# Autodesk Inventor assembly: climber
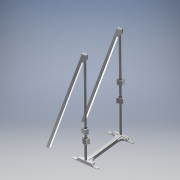
[picture p0: Inventor's stored thumbnail of the model, 180x180]
Saved by Autodesk Inventor 2019.4 (Build 234330000, 330)
## iProperties
Created: 2020-01-07
Part Number: climber
Document SubType Name: Assembly
Designer: Mark
Mass: 6066.58 g
Surface Area: 3692.19 cm^2
Volume: 1250.64 cm^3
Density: 4.85079 g/cm^3
Author: Mark
## Documents named in this file (8)
- C:\Users\Mark\Desktop\7738 Helion Engineering\7738-2020\Elevator Mechanism\climber.iam
- C:\Users\Mark\Desktop\7738 Helion Engineering\7738-2020\Elevator Mechanism\Extrusion Mid.ipt
- C:\Users\Mark\Desktop\7738 Helion Engineering\7738-2020\Elevator Mechanism\climber\Design Accelerator\Shaft2.iam
- C:\Users\Mark\Desktop\7738 Helion Engineering\7738-2020\Elevator Mechanism\scs20uu.ipt
- C:\Users\Mark\Desktop\jiagong\Base.ipt
- C:\Users\Mark\Desktop\7738 Helion Engineering\7738-2020\Elevator Mechanism\Standard Bracing.ipt
- C:\Users\Mark\Desktop\7738 Helion Engineering\7738-2020\Elevator Mechanism\Top Connector.ipt
- C:\Users\Mark\Desktop\7738 Helion Engineering\7738-2020\Elevator Mechanism\Elevator Support.ipt
## Components (17 placed, 7 different names)
1. Extrusion Mid:1 — Mate:10, Flush:3, Flush:4, Mate:12, Mate:13, Mate:16, Mate:19
2. Shaft:1 [sub-assembly] — Mate:3, Mate:4, Mate:7, Mate:8, Mate:20, Mate:21
3. Shaft:2 [sub-assembly] — Mate:1, Mate:2, Mate:6, Flush:1, Mate:26, Mate:27
4. scs20uu:1 — Mate:3
5. scs20uu:2 — Mate:1
6. scs20uu:3 — Mate:2
7. scs20uu:4 — Mate:4
8. Base:1 — Mate:6, Flush:1, Mate:9, Flush:2, Mate:10, Flush:3, Flush:4, Flush:5, Mate:11, Mate:17, Mate:18, Flush:10
9. Base:2 — Mate:7, Mate:8, Mate:9, Flush:2, Flush:5, Mate:14, Mate:15, Flush:6, Flush:7
10. Standard Bracing:1 — Mate:15, Mate:16
11. Standard Bracing:2 — Mate:13, Mate:14
12. Standard Bracing:3 — Mate:11, Mate:12
13. Standard Bracing:4 — Mate:17, Mate:18, Mate:19
14. Top Connector:1 — Mate:20, Flush:6, Mate:21, Flush:7, Mate:22, Flush:8, Mate:23
15. Elevator Support:1 — Mate:22, Flush:8, Mate:23
16. Top Connector:2 — Mate:26, Mate:27
17. Elevator Support:2 — Flush:10
## Relationships (36: Mate 26, Flush 10)
- Mate:1: Shaft:2 ↔ scs20uu:2
- Mate:2: Shaft:2 ↔ scs20uu:3
- Mate:3: Shaft:1 ↔ scs20uu:1
- Mate:4: Shaft:1 ↔ scs20uu:4
- Mate:6: Shaft:2 ↔ Base:1
- Flush:1: Shaft:2 ↔ Base:1
- Mate:7: Shaft:1 ↔ Base:2
- Mate:8: Shaft:1 ↔ Base:2
- Mate:9 (400 mm): Base:1 ↔ Base:2
- Flush:2: Base:1 ↔ Base:2
- Mate:10: Extrusion Mid:1 ↔ Base:1
- Flush:3: Extrusion Mid:1 ↔ Base:1
- Flush:4 (100 mm): Extrusion Mid:1 ↔ Base:1
- Flush:5: Base:1 ↔ Base:2
- Mate:11: Base:1 ↔ Standard Bracing:3
- Mate:12: Extrusion Mid:1 ↔ Standard Bracing:3
- Mate:13: Extrusion Mid:1 ↔ Standard Bracing:2
- Mate:14: Base:2 ↔ Standard Bracing:2
- Mate:15: Base:2 ↔ Standard Bracing:1
- Mate:16: Extrusion Mid:1 ↔ Standard Bracing:1
- Mate:17: Base:1 ↔ Standard Bracing:4
- Mate:18: Base:1 ↔ Standard Bracing:4
- Mate:19: Extrusion Mid:1 ↔ Standard Bracing:4
- Mate:20: Shaft:1 ↔ Top Connector:1
- Flush:6: Base:2 ↔ Top Connector:1
- Mate:21: Shaft:1 ↔ Top Connector:1
- Flush:7: Base:2 ↔ Top Connector:1
- Mate:22: Top Connector:1 ↔ Elevator Support:1
- Flush:8: Top Connector:1 ↔ Elevator Support:1
- Mate:23: Top Connector:1 ↔ Elevator Support:1
- [Mate]: Top Connector:2 ↔ Elevator Support:2
- [Flush]: Top Connector:2 ↔ Elevator Support:2
- [Mate]: Top Connector:2 ↔ Elevator Support:2
- Mate:26: Shaft:2 ↔ Top Connector:2
- Mate:27: Shaft:2 ↔ Top Connector:2
- Flush:10: Base:1 ↔ Elevator Support:2
## Named parameters: d41_d40 = 0 mm, d42_d38 = 0 mm, d43_d39 = 0 mm
